# Autodesk Inventor assembly: shapeoko_lowpro
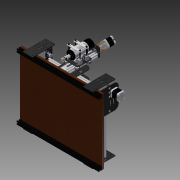
[picture p0: Inventor's stored thumbnail of the model, 180x180]
Saved by Autodesk Inventor 2014 (Build 180170000, 170)
## iProperties
Created: 2013-07-18
Part Number: shapeoko_lowpro
Document SubType Name: Assembly
Designer: Edward
Author: Edward
## Documents named in this file (10)
- C:\Users\Edward\Desktop\Shapeoko_v2.0\shapeoko_lowpro\shapeoko_lowpro.iam
- C:\Users\Edward\Desktop\Shapeoko_v2.0\shapeoko_lowpro\y_plate_assembly.iam
- C:\Users\Edward\Desktop\Shapeoko_v2.0\shapeoko_lowpro\y_plate_assembly_left.iam
- C:\Users\Edward\Desktop\Shapeoko_v2\S2_ep.ipt
- C:\Users\Edward\Documents\Shapeoko\Shapeoko_v1\Shapeoko_v1i\Shapeoko_v1i\Shapeoko v2.0\Enclosure\hfs5_2020_500.ipt
- C:\Users\Edward\Desktop\Shapeoko_v2.0\Shapeoko_bm\S2_MS400.ipt
- C:\Users\Edward\Desktop\Shapeoko_v2.0\Shapeoko_bm\two_part_wastebaord.ipt
- C:\Users\Edward\Desktop\Shapeoko_v2.0\shapeoko_lowpro\revamped_simple_z-axis_assembly.iam
- C:\Users\Edward\Desktop\Shapeoko_v2.0\shapeoko_lowpro\x_motor_assembly.iam
- C:\Users\Edward\Desktop\Shapeoko_v2.0\shapeoko_lowpro\z_mount_assembly.iam
## Components (17 placed, 9 different names)
1. S2_MS400:1 — Mate:1, Flush:1, Flush:3, Insert:10, Insert:12
2. S2_MS400:2 — Mate:2, Flush:2, Flush:3, Insert:11, Angle:2, Insert:13
3. S2_MS400:3 — Mate:15, Flush:16, Flush:20, Mate:20
4. S2_MS400:4 — Insert:2, Insert:5, Insert:6, Insert:7, Mate:16, Flush:20
5. y_plate_assembly:1 [sub-assembly] — Mate:1, Flush:1, Insert:2, Insert:5, Angle:1
6. y_plate_assembly_left:1 [sub-assembly] — Mate:2, Flush:2, Insert:6, Insert:7, Mate:20
7. S2_ep:1 — Insert:10, Angle:1, Mate:8
8. hfs5_2020_500:1 — Mate:4, Flush:6, Mate:7, Flush:10, Mate:9, Flush:11
9. S2_ep:2 — Insert:11, Angle:2, Mate:4, Flush:6, Mate:10
10. S2_ep:3 — Insert:13
11. hfs5_2020_500:2
12. S2_ep:4 — Insert:12
13. two_part_wastebaord:1 — Mate:9, Mate:10, Flush:11
14. two_part_wastebaord:2 — Mate:7, Flush:10, Mate:8
15. revamped_simple_z-axis_assembly:1 [sub-assembly] — Mate:18, Flush:18, Flush:19
16. x_motor_assembly:1 [sub-assembly] — Mate:15, Flush:16, Mate:17, Flush:17, Mate:19
17. z_mount_assembly:1 [sub-assembly] — Mate:16, Mate:17, Flush:17, Mate:18, Flush:18, Flush:19, Mate:19
## Relationships (42: Mate 16, Flush 16, Insert 8, Angle 2)
- Mate:1 (6.35 mm): S2_MS400:1 ↔ y_plate_assembly:1
- Flush:1 (-22 mm): S2_MS400:1 ↔ y_plate_assembly:1
- Mate:2 (6.35 mm): S2_MS400:2 ↔ y_plate_assembly_left:1
- Flush:2 (22 mm): S2_MS400:2 ↔ y_plate_assembly_left:1
- Insert:2: S2_MS400:4 ↔ y_plate_assembly:1
- Insert:5: S2_MS400:4 ↔ y_plate_assembly:1
- Insert:6: S2_MS400:4 ↔ y_plate_assembly_left:1
- Insert:7: S2_MS400:4 ↔ y_plate_assembly_left:1
- Flush:3: S2_MS400:1 ↔ S2_MS400:2
- [Mate]: S2_ep:1 ↔ hfs5_2020_500:1
- [Flush]: S2_ep:1 ↔ hfs5_2020_500:1
- [Flush] (-36.35 mm): S2_ep:1 ↔ hfs5_2020_500:1
- Insert:10: S2_MS400:1 ↔ S2_ep:1
- Angle:1 (0 deg): y_plate_assembly:1 ↔ S2_ep:1
- Insert:11: S2_MS400:2 ↔ S2_ep:2
- Angle:2 (0 deg): S2_MS400:2 ↔ S2_ep:2
- Mate:4: hfs5_2020_500:1 ↔ S2_ep:2
- Flush:6: hfs5_2020_500:1 ↔ S2_ep:2
- [Mate]: S2_ep:3 ↔ hfs5_2020_500:2
- [Flush]: S2_ep:3 ↔ hfs5_2020_500:2
- [Flush] (-36.35 mm): S2_ep:3 ↔ hfs5_2020_500:2
- [Mate]: hfs5_2020_500:2 ↔ S2_ep:4
- [Flush]: hfs5_2020_500:2 ↔ S2_ep:4
- Insert:12: S2_MS400:1 ↔ S2_ep:4
- Insert:13: S2_MS400:2 ↔ S2_ep:3
- Mate:7: hfs5_2020_500:1 ↔ two_part_wastebaord:2
- Flush:10: hfs5_2020_500:1 ↔ two_part_wastebaord:2
- Mate:8: S2_ep:1 ↔ two_part_wastebaord:2
- Mate:9: hfs5_2020_500:1 ↔ two_part_wastebaord:1
- Mate:10: S2_ep:2 ↔ two_part_wastebaord:1
- Flush:11: hfs5_2020_500:1 ↔ two_part_wastebaord:1
- Mate:15 (6.35 mm): S2_MS400:3 ↔ x_motor_assembly:1
- Flush:16 (-22 mm): S2_MS400:3 ↔ x_motor_assembly:1
- Mate:16 (6.35 mm): S2_MS400:4 ↔ z_mount_assembly:1
- Mate:17: x_motor_assembly:1 ↔ z_mount_assembly:1
- Flush:17: x_motor_assembly:1 ↔ z_mount_assembly:1
- Mate:18: revamped_simple_z-axis_assembly:1 ↔ z_mount_assembly:1
- Flush:18: revamped_simple_z-axis_assembly:1 ↔ z_mount_assembly:1
- Flush:19 (35 mm): revamped_simple_z-axis_assembly:1 ↔ z_mount_assembly:1
- Flush:20: S2_MS400:3 ↔ S2_MS400:4
- Mate:19 (57.15 mm): x_motor_assembly:1 ↔ z_mount_assembly:1
- Mate:20: S2_MS400:3 ↔ y_plate_assembly_left:1
## Named parameters: d26_d21 = 0 mm, d27_d22 = 0 mm, d28_d23 = 0 mm, d29_d24 = 0 mm, d30_d25 = -36.35 mm
